# Autodesk Inventor assembly: Rotado
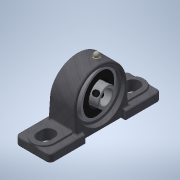
[picture p0: Inventor's stored thumbnail of the model, 180x180]
Saved by Autodesk Inventor 2021 (Build 250183000, 183)
## iProperties
Created: 2014-05-17
Part Number: Rotado
Document SubType Name: Assembly
Designer: Luis
Author: Luis
## Documents named in this file (6)
- C:\Users\79449\Documents\CNC_DISENO_DE MAQUINAS\fotos_ejemplos\chumacera-de-3-4-a-bearing.snapshot.4\Rotado.iam
- C:\Users\79449\Documents\CNC_DISENO_DE MAQUINAS\fotos_ejemplos\chumacera-de-3-4-a-bearing.snapshot.4\1Rotable.ipt
- C:\Users\79449\Documents\CNC_DISENO_DE MAQUINAS\fotos_ejemplos\chumacera-de-3-4-a-bearing.snapshot.4\2Rotable.ipt
- C:\Users\79449\Documents\CNC_DISENO_DE MAQUINAS\fotos_ejemplos\chumacera-de-3-4-a-bearing.snapshot.4\Chumacera\3.ipt
- C:\Users\79449\Documents\CNC_DISENO_DE MAQUINAS\fotos_ejemplos\chumacera-de-3-4-a-bearing.snapshot.4\Chumacera\4.ipt
- C:\Users\79449\Documents\CNC_DISENO_DE MAQUINAS\fotos_ejemplos\chumacera-de-3-4-a-bearing.snapshot.4\Chumacera\5.ipt
## Components (5 placed, 5 different names)
1. 1Rotable:1 — Mate:1, Mate:2, Mate:3, Mate:5
2. 2Rotable:1 — Mate:1, Mate:2, Mate:3, Insert:1, Mate:4
3. 3:1 — Insert:1
4. 4:1 — Mate:4
5. 5:1 — Mate:5
## Relationships (6: Mate 5, Insert 1)
- Mate:1: 1Rotable:1 ↔ 2Rotable:1
- Mate:2: 1Rotable:1 ↔ 2Rotable:1
- Mate:3: 1Rotable:1 ↔ 2Rotable:1
- Insert:1: 2Rotable:1 ↔ 3:1
- Mate:4: 2Rotable:1 ↔ 4:1
- Mate:5: 1Rotable:1 ↔ 5:1
